# Autodesk Inventor assembly: kąty
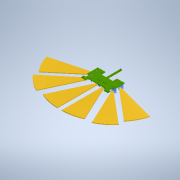
[picture p0: Inventor's stored thumbnail of the model, 180x180]
Saved by Autodesk Inventor 2022 (Build 260153000, 153)
## iProperties
Created: 2022-12-28
Part Number: kąty
Document SubType Name: Assembly
Designer: Kamil
Author: Kamil
## Documents named in this file (3)
- C:\MiniSumo koks\kąty.iam
- C:\MiniSumo koks\PCB.ipt
- C:\MiniSumo koks\TOF_VLCOS.ipt
## Components (7 placed, 2 different names)
1. PCB:1 — Mate:1, Mate:4, Mate:6, Mate:8, Mate:10, Mate:12
2. TOF_VLCOS:1 — Mate:1, Flush:1, Mate:5, Flush:2
3. TOF_VLCOS:2 — Flush:1, Mate:7, Flush:3, Mate:12
4. TOF_VLCOS:3 — Mate:4, Mate:5, Flush:2, Mate:9, Flush:4
5. TOF_VLCOS:4 — Mate:6, Mate:7, Flush:3, Mate:11, Flush:5
6. TOF_VLCOS:5 — Mate:8, Mate:9, Flush:4
7. TOF_VLCOS:6 — Mate:10, Mate:11, Flush:5
## Relationships (15: Mate 10, Flush 5)
- Mate:1: PCB:1 ↔ TOF_VLCOS:1
- Flush:1: TOF_VLCOS:1 ↔ TOF_VLCOS:2
- Mate:4: PCB:1 ↔ TOF_VLCOS:3
- Mate:5 (20 mm): TOF_VLCOS:1 ↔ TOF_VLCOS:3
- Flush:2 (8 mm): TOF_VLCOS:1 ↔ TOF_VLCOS:3
- Mate:6: PCB:1 ↔ TOF_VLCOS:4
- Mate:7 (20 mm): TOF_VLCOS:2 ↔ TOF_VLCOS:4
- Flush:3 (8 mm): TOF_VLCOS:2 ↔ TOF_VLCOS:4
- Mate:8: PCB:1 ↔ TOF_VLCOS:5
- Mate:9 (13 mm): TOF_VLCOS:3 ↔ TOF_VLCOS:5
- Flush:4 (11.5 mm): TOF_VLCOS:3 ↔ TOF_VLCOS:5
- Mate:10: PCB:1 ↔ TOF_VLCOS:6
- Mate:11 (13 mm): TOF_VLCOS:4 ↔ TOF_VLCOS:6
- Flush:5 (-11.5 mm): TOF_VLCOS:4 ↔ TOF_VLCOS:6
- Mate:12: PCB:1 ↔ TOF_VLCOS:2
